# Autodesk Inventor assembly: ensamble_goma_aro
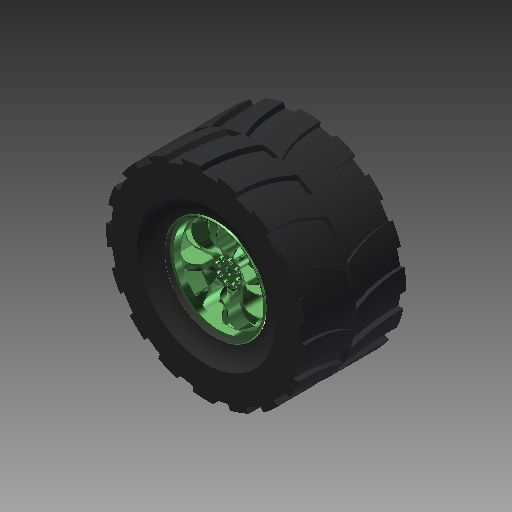
[picture p0: Inventor's stored thumbnail of the model, 512x512]
Saved by Autodesk Inventor 2017 (Build 210142000, 142)
## iProperties
Part Number: ensamble_goma_aro
Material: Genérico
Document SubType Name: Assembly
Designer: USERPC
Author: USERPC
## Documents named in this file (3)
- F:\ROBOT\ensamble_goma_aro.iam
- F:\ROBOT\llanta2.ipt
- F:\ROBOT\RIN llanta.ipt
## Components (2 placed, 2 different names)
1. llanta2:1
2. RIN llanta:1
## Relationships (1: Insert 1)
- [Insert]: llanta2:1 ↔ RIN llanta:1
